# Autodesk Inventor assembly: RCT-P011 Wheel Complete
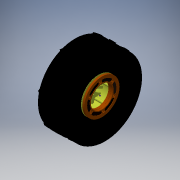
[picture p0: Inventor's stored thumbnail of the model, 180x180]
Saved by Autodesk Inventor 2019 (Build 230136000, 136)
## iProperties
Created: 2019-10-07
Part Number: RCT-P011 Wheel Complete
Material: Genérico
Document SubType Name: Assembly
Designer: david
Author: david
## Documents named in this file (4)
- C:\Users\david\OneDrive\Escritorio\RCT-P011 Wheel Complete.iam
- C:\Users\david\OneDrive\Escritorio\RCT-P010 Wheel.ipt
- C:\Users\david\OneDrive\Escritorio\RCT-P009  Rin.ipt
- C:\Users\david\OneDrive\Escritorio\RCT-H008 Wheel Frame.ipt
## Components (4 placed, 3 different names)
1. RCT-P010 Wheel:1 — Insertar:1
2. RCT-P009  Rin:1 — Insertar:1, Insertar:2, Insertar:3
3. RCT-H008 Wheel Frame:1 — Insertar:2
4. RCT-H008 Wheel Frame:2 — Insertar:3
## Relationships (3: Insert 3)
- Insertar:1: RCT-P010 Wheel:1 ↔ RCT-P009  Rin:1
- Insertar:2: RCT-P009  Rin:1 ↔ RCT-H008 Wheel Frame:1
- Insertar:3: RCT-P009  Rin:1 ↔ RCT-H008 Wheel Frame:2
